# Autodesk Inventor assembly: preview demo
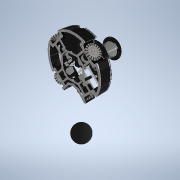
[picture p0: Inventor's stored thumbnail of the model, 180x180]
Saved by Autodesk Inventor 2020 (Build 240168000, 168)
## iProperties
Created: 2024-01-28
Part Number: preview demo
Document SubType Name: Assembly
Designer: 4s
Author: 4s
## Documents named in this file (33)
- C:\Users\4s\Documents\Inventor models\Asterisk\robot_v2\preview demo.iam
- C:\Users\4s\Documents\Inventor models\Asterisk\robot_v2\bottom_plate.ipt
- C:\Users\4s\Documents\Inventor models\Asterisk\robot_v2\motor mounts\back_motor_short.ipt
- C:\Users\4s\Documents\Inventor models\Asterisk\robot_v2\upper_plate.ipt
- C:\Users\4s\Documents\Altium projects\Asterisk TSOP Board\TSOP board 3d\tsop_board_black.iam
- C:\Users\4s\Documents\Inventor models\Asterisk\9Dof Razor IMU.ipt
- C:\Users\4s\Documents\Inventor models\Asterisk\robot_v2\kicker\kicker_base_v6_wide.ipt
- C:\Users\4s\Documents\Inventor models\Asterisk\robot_v2\kicker\kicker_head_flat_v4.ipt
- C:\Users\4s\Documents\Inventor models\Asterisk\ball.ipt
- C:\Users\4s\Documents\Inventor models\Asterisk\robot_v2\motor_body.ipt
- C:\Users\4s\Documents\Inventor models\Asterisk\robot_v2\GTF Robots 50mm Wheel.ipt
- C:\Users\4s\Documents\Inventor models\Asterisk\robot_v2\Bat_mount\bat_bed003_clear.ipt
- C:\Users\4s\Documents\Inventor models\Asterisk\robot_v2\motor mounts\right_motor_v2.ipt
- C:\Users\4s\Documents\Inventor models\Asterisk\robot_v2\openmv\openmv4_h7.iam
- C:\Users\4s\Documents\Inventor models\Asterisk\robot_v2\mirror_50.ipt
- C:\Users\4s\Documents\Inventor models\Asterisk\robot_v2\tube_50.ipt
- C:\Users\4s\Documents\Inventor models\Asterisk\robot_v2\Bat_mount\bat_sketch.ipt
- C:\Users\4s\Documents\Inventor models\Asterisk\robot_v2\upper_mount\mirror_lock_v4.ipt
- C:\Users\4s\Documents\Inventor models\Asterisk\robot_v2\board_support.ipt
- C:\Users\4s\Documents\Inventor models\Asterisk\robot_v2\upper_mount\tsop_imu_v1.ipt
- C:\Users\4s\Documents\Inventor models\Asterisk\robot_v2\upper_mount\tsop_mount_v4.ipt
- C:\Users\4s\Documents\Inventor models\Asterisk\robot_v2\side_prot.ipt
- C:\Users\4s\Documents\Inventor models\Asterisk\robot_v2\pcb_main_board\motherboard.ipt
- C:\Users\4s\Documents\Inventor models\Asterisk\robot_v2\upper_mount\optic_mount_v3.ipt
- C:\Users\4s\Documents\Inventor models\Asterisk\robot_v2\side_prot_stab_60.ipt
- C:\Users\4s\Documents\Inventor models\Asterisk\robot_v2\motor mounts\mid_mount_v3.ipt
- C:\Users\4s\Documents\Inventor models\Asterisk\robot_v2\Bat_mount\bat_case_v6.ipt
- C:\Users\4s\Documents\Inventor models\Asterisk\robot_v2\motor mounts\left_motor_v3.ipt
- C:\Users\4s\Documents\Inventor models\Asterisk\robot_v2\main2\AIP\FEA\enhbkxbnk.fins
- C:\Users\4s\Documents\Inventor models\Asterisk\robot_v2\main2\AIP\FEA\enhbkxbog.fsat
- C:\Users\4s\Documents\Inventor models\Asterisk\robot_v2\main2\AIP\FEA\enhbkxbog.ftes
- C:\Users\4s\Documents\Inventor models\Asterisk\robot_v2\main2\AIP\FEA\enhbkxbog.fwiz
- C:\Users\4s\Documents\Inventor models\Asterisk\robot_v2\main2\AIP\FEA\enhbkxl1c.fmsh
## Components (37 placed, 27 different names)
1. bottom_plate:1 — Совмещение:1, Совмещение:2, Совмещение:3, Совмещение:10, Совмещение:11, Совмещение:12, Совмещение:13, Совмещение:14, Совмещение:15, Совмещение:46, Совмещение:47, Совмещение:48, Совмещение:100, Совмещение:101, Совмещение:102, Совмещение:109, Совмещение:110, Совмещение:111, Совмещение:179, Совмещение:180, Совмещение:181, Совмещение:195, Совмещение:197, Совмещение:199, Совмещение:200, Совмещение:201, Совмещение:203, Совмещение:205, Совмещение:207, Совмещение:209, Совмещение:210, Совмещение:211, Совмещение:212
2. back_motor_short:1 — Совмещение:13, Совмещение:14, Совмещение:15, Совмещение:80, Совмещение:87, Совмещение:95, Совмещение:103, Совмещение:104
3. back_motor_short:2 — Совмещение:10, Совмещение:11, Совмещение:12, Совмещение:83, Совмещение:84, Совмещение:85, Совмещение:93
4. upper_plate:1 — Совмещение:103, Совмещение:104, Совмещение:125, Совмещение:127, Совмещение:161, Совмещение:162, Совмещение:163, Совмещение:173, Совмещение:174, Совмещение:184, Совмещение:189
5. 9Dof Razor IMU:1 — Совмещение:24, Угол:2, Совмещение:172
6. kicker_base_v6_wide:1 — Совмещение:46, Совмещение:47, Совмещение:48, Совмещение:61, Совмещение:62, Совмещение:63, Совмещение:67
7. kicker_head_flat_v4:1 — Совмещение:61, Совмещение:62, Совмещение:63, Совмещение:67
8. ball:1 — Совмещение:65, Совмещение:66
9. motor_body:1 — Совмещение:80, Совмещение:87, Совмещение:89, Совмещение:206
10. motor_body:2 — Совмещение:91, Совмещение:202
11. motor_body:3 — Совмещение:90, Совмещение:112, Совмещение:113, Совмещение:114, Совмещение:198
12. motor_body:4 — Совмещение:83, Совмещение:84, Совмещение:85, Совмещение:92, Совмещение:204
13. GTF Robots 50mm Wheel:1 — Совмещение:90, Совмещение:115
14. GTF Robots 50mm Wheel:2 — Совмещение:91
15. GTF Robots 50mm Wheel:3 — Совмещение:92, Совмещение:93
16. GTF Robots 50mm Wheel:4 — Совмещение:89, Совмещение:95
17. bat_bed003_clear:1 — Совмещение:100, Совмещение:101, Совмещение:102, Совмещение:208
18. right_motor_v2:1 — Совмещение:109, Совмещение:110, Совмещение:111, Совмещение:112, Совмещение:113, Совмещение:114, Совмещение:115
19. tsop_board_black:1 [sub-assembly] — Заподлицо:4, Угол:7
20. openmv4_h7:1 [sub-assembly] — Угол:9, Угол:10, Совмещение:136, Совмещение:192
21. mirror_50:1 — Угол:11, Совмещение:135, Совмещение:136, Совмещение:158, Совмещение:191
22. bat_sketch:1 — Угол:15
23. mirror_lock_v4:1 — Совмещение:158, Совмещение:191
24. board_support:1 — Совмещение:161, Совмещение:162, Совмещение:163, Совмещение:182, Совмещение:183
25. tsop_imu_v1:1 — Совмещение:172, Совмещение:175, Совмещение:186, Совмещение:187, Совмещение:188, Совмещение:190
26. tsop_mount_v4:1 — Совмещение:173, Совмещение:174, Совмещение:175, Совмещение:188, Совмещение:189
27. side_prot:2 — Совмещение:179, Совмещение:180, Совмещение:181, Совмещение:207
28. motherboard:1 — Совмещение:182, Совмещение:183, Совмещение:184
29. optic_mount_v3:1 — Совмещение:186, Совмещение:187, Совмещение:192, Совмещение:213, Совмещение:214
30. side_prot_stab_60:1 — Совмещение:195
31. mid_mount_v3:1 — Совмещение:197, Совмещение:198, Совмещение:199
32. mid_mount_v3:2 — Совмещение:200, Совмещение:201, Совмещение:202
33. mid_mount_v3:3 — Совмещение:203, Совмещение:204
34. mid_mount_v3:4 — Совмещение:205, Совмещение:206
35. bat_case_v6:1 — Совмещение:208, Заподлицо:6, Совмещение:209
36. left_motor_v3:1 — Совмещение:210, Совмещение:211, Совмещение:212
37. tube_50:1 — Совмещение:213, Совмещение:214
## Relationships (97: Mate 88, Angle 6, Flush 3)
- Совмещение:1 [Mate] (9 mm): bottom_plate:1
- Совмещение:2 [Mate]: bottom_plate:1
- Совмещение:3 [Mate]: bottom_plate:1
- Совмещение:10 [Mate]: bottom_plate:1 ↔ back_motor_short:2
- Совмещение:11 [Mate]: bottom_plate:1 ↔ back_motor_short:2
- Совмещение:12 [Mate]: bottom_plate:1 ↔ back_motor_short:2
- Совмещение:13 [Mate]: bottom_plate:1 ↔ back_motor_short:1
- Совмещение:14 [Mate]: bottom_plate:1 ↔ back_motor_short:1
- Совмещение:15 [Mate]: bottom_plate:1 ↔ back_motor_short:1
- Совмещение:24 [Mate]: 9Dof Razor IMU:1
- Угол:2 [Angle] (0 deg): 9Dof Razor IMU:1
- Совмещение:46 [Mate]: bottom_plate:1 ↔ kicker_base_v6_wide:1
- Совмещение:47 [Mate]: bottom_plate:1 ↔ kicker_base_v6_wide:1
- Совмещение:48 [Mate]: bottom_plate:1 ↔ kicker_base_v6_wide:1
- Совмещение:61 [Mate]: kicker_base_v6_wide:1 ↔ kicker_head_flat_v4:1
- Совмещение:62 [Mate]: kicker_base_v6_wide:1 ↔ kicker_head_flat_v4:1
- Совмещение:63 [Mate]: kicker_base_v6_wide:1 ↔ kicker_head_flat_v4:1
- Совмещение:65 [Mate]: ball:1
- Совмещение:66 [Mate] (37 mm): ball:1
- Совмещение:67 [Mate]: kicker_base_v6_wide:1 ↔ kicker_head_flat_v4:1
- Совмещение:80 [Mate]: back_motor_short:1 ↔ motor_body:1
- Совмещение:83 [Mate]: back_motor_short:2 ↔ motor_body:4
- Совмещение:84 [Mate]: back_motor_short:2 ↔ motor_body:4
- Совмещение:85 [Mate]: back_motor_short:2 ↔ motor_body:4
- Совмещение:87 [Mate]: back_motor_short:1 ↔ motor_body:1
- Совмещение:89 [Mate]: motor_body:1 ↔ GTF Robots 50mm Wheel:4
- Совмещение:90 [Mate]: motor_body:3 ↔ GTF Robots 50mm Wheel:1
- Совмещение:91 [Mate]: motor_body:2 ↔ GTF Robots 50mm Wheel:2
- Совмещение:92 [Mate]: motor_body:4 ↔ GTF Robots 50mm Wheel:3
- Совмещение:93 [Mate] (1 mm): back_motor_short:2 ↔ GTF Robots 50mm Wheel:3
- Совмещение:95 [Mate] (1 mm): back_motor_short:1 ↔ GTF Robots 50mm Wheel:4
- Заподлицо:3 [Flush] (220 mm)
- Совмещение:100 [Mate]: bottom_plate:1 ↔ bat_bed003_clear:1
- Совмещение:101 [Mate]: bottom_plate:1 ↔ bat_bed003_clear:1
- Совмещение:102 [Mate]: bottom_plate:1 ↔ bat_bed003_clear:1
- Совмещение:103 [Mate]: back_motor_short:1 ↔ upper_plate:1
- Совмещение:104 [Mate]: back_motor_short:1 ↔ upper_plate:1
- Совмещение:109 [Mate]: bottom_plate:1 ↔ right_motor_v2:1
- Совмещение:110 [Mate]: bottom_plate:1 ↔ right_motor_v2:1
- Совмещение:111 [Mate]: bottom_plate:1 ↔ right_motor_v2:1
- Совмещение:112 [Mate]: motor_body:3 ↔ right_motor_v2:1
- Совмещение:113 [Mate]: motor_body:3 ↔ right_motor_v2:1
- Совмещение:114 [Mate]: motor_body:3 ↔ right_motor_v2:1
- Совмещение:115 [Mate] (1 mm): GTF Robots 50mm Wheel:1 ↔ right_motor_v2:1
- Заподлицо:4 [Flush]: tsop_board_black:1
- Угол:7 [Angle] (180 deg): tsop_board_black:1
- Угол:9 [Angle] (180 deg): openmv4_h7:1
- Угол:10 [Angle] (180 deg): openmv4_h7:1
- Угол:11 [Angle] (0 deg): mirror_50:1
- Совмещение:125 [Mate]: upper_plate:1
- Совмещение:127 [Mate]: upper_plate:1
- Совмещение:129 [Mate]
- Совмещение:130 [Mate]
- Совмещение:135 [Mate]: mirror_50:1
- Совмещение:136 [Mate] (30 mm): openmv4_h7:1 ↔ mirror_50:1
- Угол:15 [Angle] (0 deg): bat_sketch:1
- Совмещение:158 [Mate]: mirror_50:1 ↔ mirror_lock_v4:1
- Совмещение:161 [Mate]: upper_plate:1 ↔ board_support:1
- Совмещение:162 [Mate]: upper_plate:1 ↔ board_support:1
- Совмещение:163 [Mate]: upper_plate:1 ↔ board_support:1
- Совмещение:172 [Mate]: 9Dof Razor IMU:1 ↔ tsop_imu_v1:1
- Совмещение:173 [Mate]: upper_plate:1 ↔ tsop_mount_v4:1
- Совмещение:174 [Mate]: upper_plate:1 ↔ tsop_mount_v4:1
- Совмещение:175 [Mate]: tsop_imu_v1:1 ↔ tsop_mount_v4:1
- Совмещение:179 [Mate]: bottom_plate:1 ↔ side_prot:2
- Совмещение:180 [Mate]: bottom_plate:1 ↔ side_prot:2
- Совмещение:181 [Mate]: bottom_plate:1 ↔ side_prot:2
- Совмещение:182 [Mate]: board_support:1 ↔ motherboard:1
- Совмещение:183 [Mate]: board_support:1 ↔ motherboard:1
- Совмещение:184 [Mate]: upper_plate:1 ↔ motherboard:1
- Совмещение:186 [Mate]: tsop_imu_v1:1 ↔ optic_mount_v3:1
- Совмещение:187 [Mate]: tsop_imu_v1:1 ↔ optic_mount_v3:1
- Совмещение:188 [Mate]: tsop_imu_v1:1 ↔ tsop_mount_v4:1
- Совмещение:189 [Mate]: upper_plate:1 ↔ tsop_mount_v4:1
- Совмещение:190 [Mate]: tsop_imu_v1:1
- Совмещение:191 [Mate]: mirror_50:1 ↔ mirror_lock_v4:1
- Совмещение:192 [Mate]: openmv4_h7:1 ↔ optic_mount_v3:1
- Совмещение:195 [Mate]: bottom_plate:1 ↔ side_prot_stab_60:1
- Совмещение:197 [Mate]: bottom_plate:1 ↔ mid_mount_v3:1
- Совмещение:198 [Mate]: motor_body:3 ↔ mid_mount_v3:1
- Совмещение:199 [Mate]: bottom_plate:1 ↔ mid_mount_v3:1
- Совмещение:200 [Mate]: bottom_plate:1 ↔ mid_mount_v3:2
- Совмещение:201 [Mate]: bottom_plate:1 ↔ mid_mount_v3:2
- Совмещение:202 [Mate]: motor_body:2 ↔ mid_mount_v3:2
- Совмещение:203 [Mate]: bottom_plate:1 ↔ mid_mount_v3:3
- Совмещение:204 [Mate]: motor_body:4 ↔ mid_mount_v3:3
- Совмещение:205 [Mate]: bottom_plate:1 ↔ mid_mount_v3:4
- Совмещение:206 [Mate]: motor_body:1 ↔ mid_mount_v3:4
- Совмещение:207 [Mate]: bottom_plate:1 ↔ side_prot:2
- Совмещение:208 [Mate]: bat_bed003_clear:1 ↔ bat_case_v6:1
- Заподлицо:6 [Flush]: bat_case_v6:1
- Совмещение:209 [Mate]: bottom_plate:1 ↔ bat_case_v6:1
- Совмещение:210 [Mate]: bottom_plate:1 ↔ left_motor_v3:1
- Совмещение:211 [Mate]: bottom_plate:1 ↔ left_motor_v3:1
- Совмещение:212 [Mate]: bottom_plate:1 ↔ left_motor_v3:1
- Совмещение:213 [Mate]: optic_mount_v3:1 ↔ tube_50:1
- Совмещение:214 [Mate]: optic_mount_v3:1 ↔ tube_50:1
## Named parameters: sa_0 = 98268.7, sa_1 = -2.838e-10, sa_2 = 18527.3
note: some values were not read from the file. Shown as the stored number, unit unknown: "sa_0", "sa_1", "sa_2".
